# Autodesk Inventor assembly: Montagem Prensa e suporte coletor
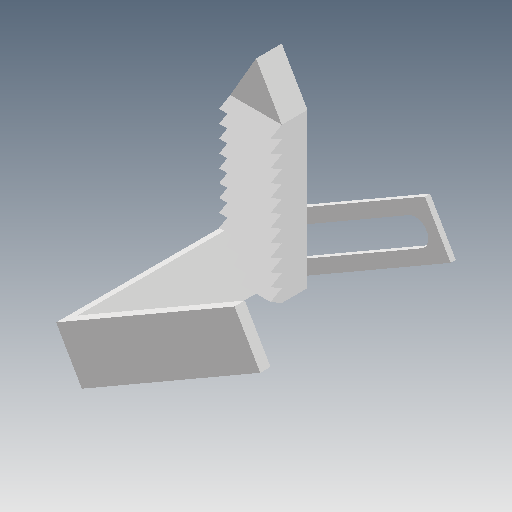
[picture p0: Inventor's stored thumbnail of the model, 512x512]
Saved by Autodesk Inventor 2021 (Build 250183000, 183)
## iProperties
Created: 2020-09-23
Part Number: Montagem Prensa e suporte coletor
Document SubType Name: Assembly
Designer: rapha
Author: rapha
## Documents named in this file (3)
- C:\Users\evert\OneDrive\Área de Trabalho\peca move\coleotr\Montagem_Prensa_e_suporte_coletor.iam
- C:\Users\evert\OneDrive\Área de Trabalho\peca move\coleotr\Suporte_prensas_coletor.ipt
- C:\Users\evert\OneDrive\Área de Trabalho\peca move\coleotr\Prensas_coletor.ipt
## Components (2 placed, 2 different names)
1. Suporte_prensas_coletor:1 — Rígida:1
2. Prensas_coletor:1 — Rígida:1
## Relationships (1: WeldJoint 1)
- Rígida:1 [WeldJoint]: Suporte_prensas_coletor:1 ↔ Prensas_coletor:1
